# Autodesk Inventor assembly: Assembly1
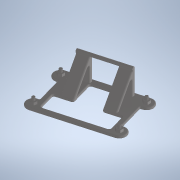
[picture p0: Inventor's stored thumbnail of the model, 180x180]
Saved by Autodesk Inventor 2020.3 (Build 243373000, 373)
## iProperties
Created: 2020-08-29
Part Number: Assembly1
Document SubType Name: Assembly
Designer: franc
Author: franc
## Documents named in this file (4)
- D:\progetti kicad\PSE\PSE_BOARD_ESP32_ALL_IN1PCB\3Dfile\ALL_ASEMBLED_SUPPORT_OLED\Assembly1.iam
- D:\progetti kicad\PSE\PSE_BOARD_ESP32_ALL_IN1PCB\3Dfile\M3 Nut.ipt
- D:\progetti kicad\PSE\PSE_BOARD_ESP32_ALL_IN1PCB\3Dfile\screw M3 6mm .ipt
- D:\progetti kicad\PSE\PSE_BOARD_ESP32_ALL_IN1PCB\3Dfile\suppotoOLED.ipt
## Components (9 placed, 3 different names)
1. M3 Nut:1 — Mate:1, Flush:1, Flush:2
2. screw M3 6mm :1 — Flush:4, Flush:5, Mate:6
3. suppotoOLED:1 — Mate:1, Mate:2, Mate:3, Mate:4, Mate:5, Flush:7, Mate:6, Mate:7, Mate:8, Mate:9
4. M3 Nut:2 — Mate:2, Flush:2, Flush:3, Mate:5
5. screw M3 6mm :2 — Flush:4, Mate:9
6. M3 Nut:3 — Mate:3, Flush:3
7. screw M3 6mm :3 — Flush:5, Flush:6, Flush:7, Mate:7
8. M3 Nut:4 — Mate:4, Flush:1
9. screw M3 6mm :4 — Flush:6, Mate:8
## Relationships (16: Mate 9, Flush 7)
- Mate:1: M3 Nut:1 ↔ suppotoOLED:1
- Mate:2: suppotoOLED:1 ↔ M3 Nut:2
- Mate:3: suppotoOLED:1 ↔ M3 Nut:3
- Mate:4: suppotoOLED:1 ↔ M3 Nut:4
- Flush:1: M3 Nut:1 ↔ M3 Nut:4
- Flush:2: M3 Nut:1 ↔ M3 Nut:2
- Flush:3: M3 Nut:2 ↔ M3 Nut:3
- Mate:5: suppotoOLED:1 ↔ M3 Nut:2
- Flush:4: screw M3 6mm :1 ↔ screw M3 6mm :2
- Flush:5: screw M3 6mm :1 ↔ screw M3 6mm :3
- Flush:6: screw M3 6mm :3 ↔ screw M3 6mm :4
- Flush:7: suppotoOLED:1 ↔ screw M3 6mm :3
- Mate:6: screw M3 6mm :1 ↔ suppotoOLED:1
- Mate:7: suppotoOLED:1 ↔ screw M3 6mm :3
- Mate:8: suppotoOLED:1 ↔ screw M3 6mm :4
- Mate:9: suppotoOLED:1 ↔ screw M3 6mm :2
